# Autodesk Inventor assembly: 04-0008
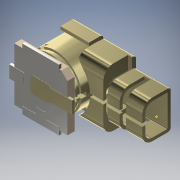
[picture p0: Inventor's stored thumbnail of the model, 180x180]
Saved by Autodesk Inventor 2018 (Build 220112000, 112)
## iProperties
Created: 2019-09-21
Part Number: 04-0008
Document SubType Name: Assembly
Designer: Bradley
Author: Bradley
## Documents named in this file (3)
- C:\Users\Bradley\Documents\GitHub\Resources\SupplierDocuments\04 - Connectors SMT\04-0008\04-0008.iam
- C:\Users\Bradley\Documents\GitHub\Resources\SupplierDocuments\04 - Connectors SMT\04-0008\04-0008.ipt
- C:\Users\Bradley\Documents\GitHub\Resources\SupplierDocuments\04 - Connectors SMT\04-0008\04-0008P.ipt
## Components (2 placed, 2 different names)
1. 04-0008:1 — Insert:1
2. 04-0008P:1 — Insert:1
## Relationships (1: Insert 1)
- Insert:1: 04-0008:1 ↔ 04-0008P:1
